# Autodesk Inventor assembly: PCB Stack Concept V03 01
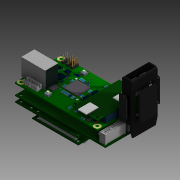
[picture p0: Inventor's stored thumbnail of the model, 180x180]
Saved by Autodesk Inventor 2013 (Build 170138000, 138)
## iProperties
Created: 2014-04-13
Part Number: PCB Stack Concept V03 01
Document SubType Name: Assembly
Designer: spichelh
Author: spichelh
## Documents named in this file (37)
- C:\Users\spichelh\Documents\GitHub\beta-hardware\Enclosure\Version 002\PCB Stack Concept V03 01.iam
- C:\Users\spichelh\Documents\GitHub\beta-hardware\Enclosure\Version 002\Enclosure-Backplate01.ipt
- C:\Users\spichelh\Documents\GitHub\beta-hardware\Enclosure\Version 002\KAC12040.ipt
- C:\Users\spichelh\Documents\GitHub\beta-hardware\Enclosure\Version 002\IRGlass.ipt
- C:\Users\spichelh\Documents\GitHub\beta-hardware\Enclosure\Version 002\Cooler.ipt
- C:\Users\spichelh\Documents\GitHub\beta-hardware\Enclosure\Version 002\Nikon Mount 02.ipt
- C:\Users\spichelh\Documents\GitHub\beta-hardware\Enclosure\Version 002\IOModulePlate01.ipt
- C:\Users\spichelh\Documents\GitHub\beta-hardware\Enclosure\Version 002\PCBModuleLeft01.ipt
- C:\Users\spichelh\Documents\GitHub\beta-hardware\Enclosure\Version 002\IOModulePlate02.ipt
- C:\Users\spichelh\Documents\GitHub\beta-hardware\Enclosure\Version 002\IOModulePlate03.ipt
- C:\Users\spichelh\Documents\GitHub\beta-hardware\Enclosure\Version 002\PCBModuleRight01.ipt
- C:\Users\spichelh\Documents\GitHub\beta-hardware\Enclosure\Version 002\LensBase02.ipt
- C:\Users\spichelh\Documents\GitHub\beta-hardware\Enclosure\Version 002\HexSaver01.ipt
- C:\Users\spichelh\Documents\GitHub\beta-hardware\Enclosure\Version 002\Enclosure03.ipt
- C:\Users\spichelh\Documents\Inventor\Content Center Files\R2013\en-US\ANSI B18.3.1M(1)\ANSI B18.3.1M - M2,5x0,45 x 16(2).ipt
- C:\Users\spichelh\Documents\Inventor\Content Center Files\R2013\en-US\ANSI B18.3.1M(1)\ANSI B18.3.1M - M2,5x0,45 x 35(2).ipt
- C:\Users\spichelh\Documents\GitHub\beta-hardware\Enclosure\Version 002\LensBaseTop01.ipt
- C:\Users\spichelh\Documents\Inventor\Content Center Files\R2013\en-US\ANSI B18.6.3(00)\ANSI B18.6.3 - 3-48 UNC - 0,25(32).ipt
- C:\Users\spichelh\Documents\GitHub\beta-hardware\Enclosure\Version 002\Unmate01.ipt
- C:\Users\spichelh\Documents\GitHub\beta-hardware\Enclosure\Version 002\Parallella.ipt
- C:\Users\spichelh\Documents\GitHub\beta-hardware\Enclosure\Version 002\SFE-Host01.ipt
- C:\Users\spichelh\Documents\GitHub\beta-hardware\Enclosure\Version 002\SFE-ProcessingBoard01.ipt
- C:\Users\spichelh\Documents\GitHub\beta-hardware\Enclosure\Version 002\CMV12000.ipt
- C:\Users\spichelh\Documents\GitHub\beta-hardware\Enclosure\Version 002\Enclosure-Backplate-Variant02.ipt
- C:\Users\spichelh\Documents\GitHub\beta-hardware\Enclosure\Version 002\PCBModuleLeft02.ipt
- C:\Users\spichelh\Documents\GitHub\beta-hardware\Enclosure\Version 002\BetaBoard01.ipt
- C:\Users\spichelh\Documents\GitHub\beta-hardware\Enclosure\Version 002\Imported Components\Zynq_Z010_uZed_F_Prod\Zynq_Z010_uZed_F_Prod.ipt
- C:\Users\spichelh\Documents\GitHub\beta-hardware\Enclosure\Version 002\HighSpeedIOShield01.ipt
- C:\Users\spichelh\Documents\GitHub\beta-hardware\Enclosure\Version 002\AddonPCB01.ipt
- C:\Users\spichelh\Documents\GitHub\beta-hardware\Enclosure\Version 002\Imported Components\PCI-E x1\PCI-E x1.ipt
- C:\Users\spichelh\Desktop\BetaSkeletonV01.ipt
- C:\Users\spichelh\Documents\GitHub\alpha-hardware\Nikon-F-Mount\Imported Components\F-mount to CMV12k-V04\F-mount to CMV12k-V04.ipt
- C:\Users\spichelh\Desktop\Imported Components\User Library-Mini Displayport Molex-sd-105081-001\User Library-Mini Displayport Molex-sd-105081-001.ipt
- C:\Users\spichelh\Documents\GitHub\beta-hardware\Enclosure\Version 002\DictatorEnclosure4.ipt
- C:\Users\spichelh\Documents\GitHub\beta-hardware\Enclosure\Version 002\IO-Shield-Sideplate01.ipt
- C:\Users\spichelh\Documents\Inventor\Content Center Files\R2013\en-US\ANSI B18.6.3(25)\ANSI B18.6.3 - 2-56 UNC - 0,125(5).ipt
- C:\Users\spichelh\Documents\GitHub\beta-hardware\Enclosure\Version 002\IO-Shield-Topplate01.ipt
## Components (55 placed, 36 different names)
1. Enclosure03:1 — Flush:26, Mate:33, Mate:34, Mate:38, Flush:40, Insert:9, Insert:10, Insert:11, Insert:13, Insert:14, Insert:27, Insert:28, Insert:29, Mate:70, Mate:71, Flush:46, Flush:47
2. Enclosure-Backplate01:1 — Mate:38, Flush:40, Mate:75
3. KAC12040:1 — Mate:72
4. IRGlass:1 — Mate:50, Mate:51, Mate:52
5. Cooler:1 — Mate:35, Flush:43, Flush:44, Mate:67, Mate:68, Mate:69
6. Nikon Mount 02:1 — Mate:31, Mate:32, Insert:3, Mate:50, Mate:51, Mate:52, Insert:18, Insert:19, Insert:20, Insert:21
7. LensBase02:1 — Mate:31, Mate:32, Flush:26, Mate:33, Mate:34, Insert:3, Mate:35, Flush:43, Flush:44, Flush:45
8. IOModulePlate01:1 — Insert:13, Insert:14
9. PCBModuleLeft01:1
10. PCBModuleRight01:1
11. IOModulePlate02:1 — Insert:11
12. IOModulePlate03:1 — Insert:9, Insert:10
13. HexSaver01:1
14. HexSaver01:2
15. HexSaver01:3
16. HexSaver01:4
17. Broached Socket Head Cap Screw - Metric M2,5x0,45 x 16:1 — Insert:18
18. Broached Socket Head Cap Screw - Metric M2,5x0,45 x 16:2 — Insert:19
19. Broached Socket Head Cap Screw - Metric M2,5x0,45 x 16:3 — Insert:20
20. Broached Socket Head Cap Screw - Metric M2,5x0,45 x 16:4 — Insert:21
21. LensBaseTop01:1 — Flush:45, Mate:53, Mate:54, Mate:67, Mate:68, Mate:69
22. Cross Recessed 100° Flat Countersunk Head Machine Screw - Type I - Inch 3-48 UNC x 0,25:2 — Mate:53
23. Cross Recessed 100° Flat Countersunk Head Machine Screw - Type I - Inch 3-48 UNC x 0,25:1 — Mate:54
24. Broached Socket Head Cap Screw - Metric M2,5x0,45 x 35:5 — Mate:55, Mate:70, Mate:71
25. Broached Socket Head Cap Screw - Metric M2,5x0,45 x 35:6 — Insert:27, Mate:59
26. Broached Socket Head Cap Screw - Metric M2,5x0,45 x 35:7 — Insert:28, Mate:66
27. Broached Socket Head Cap Screw - Metric M2,5x0,45 x 35:8 — Insert:29, Mate:57
28. Unmate01:1 — Mate:55
29. Unmate01:2 — Mate:57
30. Unmate01:3 — Mate:59
31. Unmate01:4 — Mate:66
32. Parallella:1
33. SFE-Host01:1 — Mate:72, Mate:73, Flush:48, Flush:49, Mate:76, Flush:50, Flush:51, Flush:78
34. SFE-ProcessingBoard01:1 — Mate:73, Flush:48, Flush:49, Mate:77, Flush:85
35. CMV12000:1 — Mate:76, Flush:50, Flush:51, Mate:91, Mate:92, Mate:93
36. Enclosure-Backplate-Variant02:1 — Mate:75, Flush:46, Flush:47
37. PCBModuleLeft02:1 — Flush:52, Flush:79, Mate:79
38. BetaBoard01:1 — Mate:77, Flush:52, Flush:78, Flush:79, Mate:79, Flush:85, Flush:86, Flush:87, Mate:80, Flush:88, Mate:84, Mate:85, Flush:94, Flush:95, Flush:96, Flush:97
39. Zynq_Z010_uZed_F_Prod:1 — Flush:86, Flush:87, Mate:80, Flush:91, Mate:83, Flush:92
40. HighSpeedIOShield01:1 — Flush:88, Mate:86, Mate:87, Mate:97, Mate:98, Mate:99, Flush:100, Mate:100, Mate:102, Mate:103, Mate:104, Mate:113, Mate:114, Mate:115, Mate:116, Mate:117, Mate:118, Mate:119, Mate:120, Mate:121, Mate:122, Mate:123, Mate:124, Mate:125, Mate:126
41. AddonPCB01:1 — Flush:91, Mate:83, Flush:92
42. PCI-E x1:1 — Mate:84, Flush:94, Flush:97, Mate:86, Mate:87
43. PCI-E x1:2 — Mate:85, Flush:95, Flush:96
44. BetaSkeletonV01:1 — Mate:94, Mate:95, Mate:96, Mate:39
45. F-mount to CMV12k-V04:1 — Mate:91, Mate:92, Mate:93, Mate:94, Mate:95, Mate:96
46. User Library-Mini Displayport Molex-sd-105081-001:1 — Mate:99, Flush:100, Mate:101, Mate:102, Flush:101
47. DictatorEnclosure4:1 — Mate:97, Mate:98
48. User Library-Mini Displayport Molex-sd-105081-001:2 — Mate:100, Mate:101, Flush:101
49. IO-Shield-Sideplate01:1 — Mate:103, Mate:104
50. Cross Recessed Pan Head Machine Screw - Type IA - Inch No. 2 - 56 - 1/8:1 — Mate:113, Mate:114
51. Cross Recessed Pan Head Machine Screw - Type IA - Inch No. 2 - 56 - 1/8:2 — Mate:115, Mate:116
52. Cross Recessed Pan Head Machine Screw - Type IA - Inch No. 2 - 56 - 1/8:3 — Mate:117, Mate:118
53. Cross Recessed Pan Head Machine Screw - Type IA - Inch No. 2 - 56 - 1/8:4 — Mate:119, Mate:120
54. IO-Shield-Topplate01:1 — Mate:124, Mate:125, Mate:126
55. IO-Shield-Topplate01:2 — Mate:121, Mate:122, Mate:123
## Relationships (100: Mate 61, Flush 26, Insert 13)
- Mate:31: Nikon Mount 02:1 ↔ LensBase02:1
- Mate:32: Nikon Mount 02:1 ↔ LensBase02:1
- Flush:26: Enclosure03:1 ↔ LensBase02:1
- Mate:33: Enclosure03:1 ↔ LensBase02:1
- Mate:34: Enclosure03:1 ↔ LensBase02:1
- Insert:3: Nikon Mount 02:1 ↔ LensBase02:1
- Mate:35: Cooler:1 ↔ LensBase02:1
- Mate:38 (3 mm): Enclosure03:1 ↔ Enclosure-Backplate01:1
- Flush:40: Enclosure03:1 ↔ Enclosure-Backplate01:1
- Mate:39: BetaSkeletonV01:1
- Insert:9: Enclosure03:1 ↔ IOModulePlate03:1
- Insert:10: Enclosure03:1 ↔ IOModulePlate03:1
- Insert:11: Enclosure03:1 ↔ IOModulePlate02:1
- Insert:13: Enclosure03:1 ↔ IOModulePlate01:1
- Insert:14: Enclosure03:1 ↔ IOModulePlate01:1
- Mate:50: IRGlass:1 ↔ Nikon Mount 02:1
- Mate:51 (0.5 mm): IRGlass:1 ↔ Nikon Mount 02:1
- Mate:52 (0.5 mm): IRGlass:1 ↔ Nikon Mount 02:1
- Flush:43: Cooler:1 ↔ LensBase02:1
- Flush:44: Cooler:1 ↔ LensBase02:1
- Flush:45: LensBase02:1 ↔ LensBaseTop01:1
- Mate:55: Broached Socket Head Cap Screw - Metric M2,5x0,45 x 35:5 ↔ Unmate01:1
- Mate:57: Broached Socket Head Cap Screw - Metric M2,5x0,45 x 35:8 ↔ Unmate01:2
- Mate:59: Broached Socket Head Cap Screw - Metric M2,5x0,45 x 35:6 ↔ Unmate01:3
- Mate:66: Broached Socket Head Cap Screw - Metric M2,5x0,45 x 35:7 ↔ Unmate01:4
- Mate:67: Cooler:1 ↔ LensBaseTop01:1
- Mate:68: Cooler:1 ↔ LensBaseTop01:1
- Mate:69: Cooler:1 ↔ LensBaseTop01:1
- Mate:70: Enclosure03:1 ↔ Broached Socket Head Cap Screw - Metric M2,5x0,45 x 35:5
- Mate:71: Enclosure03:1 ↔ Broached Socket Head Cap Screw - Metric M2,5x0,45 x 35:5
- Mate:72: KAC12040:1 ↔ SFE-Host01:1
- Mate:73: SFE-Host01:1 ↔ SFE-ProcessingBoard01:1
- Mate:75 (10 mm): Enclosure-Backplate01:1 ↔ Enclosure-Backplate-Variant02:1
- Flush:46: Enclosure03:1 ↔ Enclosure-Backplate-Variant02:1
- Flush:47: Enclosure03:1 ↔ Enclosure-Backplate-Variant02:1
- Flush:48: SFE-Host01:1 ↔ SFE-ProcessingBoard01:1
- Flush:49: SFE-Host01:1 ↔ SFE-ProcessingBoard01:1
- Mate:76 (3 mm): SFE-Host01:1 ↔ CMV12000:1
- Flush:50 (6 mm): SFE-Host01:1 ↔ CMV12000:1
- Flush:51 (11.75 mm): SFE-Host01:1 ↔ CMV12000:1
- Mate:77: SFE-ProcessingBoard01:1 ↔ BetaBoard01:1
- Flush:52: PCBModuleLeft02:1 ↔ BetaBoard01:1
- Flush:78: SFE-Host01:1 ↔ BetaBoard01:1
- Flush:79: PCBModuleLeft02:1 ↔ BetaBoard01:1
- Mate:79 (6 mm): PCBModuleLeft02:1 ↔ BetaBoard01:1
- Flush:85 (-21 mm): SFE-ProcessingBoard01:1 ↔ BetaBoard01:1
- Flush:86: BetaBoard01:1 ↔ Zynq_Z010_uZed_F_Prod:1
- Flush:87: BetaBoard01:1 ↔ Zynq_Z010_uZed_F_Prod:1
- Mate:80 (12 mm): BetaBoard01:1 ↔ Zynq_Z010_uZed_F_Prod:1
- Flush:88: BetaBoard01:1 ↔ HighSpeedIOShield01:1
- Flush:91: Zynq_Z010_uZed_F_Prod:1 ↔ AddonPCB01:1
- Mate:83: Zynq_Z010_uZed_F_Prod:1 ↔ AddonPCB01:1
- Flush:92: Zynq_Z010_uZed_F_Prod:1 ↔ AddonPCB01:1
- Mate:84: BetaBoard01:1 ↔ PCI-E x1:1
- Mate:85: BetaBoard01:1 ↔ PCI-E x1:2
- Flush:94 (2 mm): BetaBoard01:1 ↔ PCI-E x1:1
- Flush:95 (2 mm): BetaBoard01:1 ↔ PCI-E x1:2
- Flush:96 (2 mm): BetaBoard01:1 ↔ PCI-E x1:2
- Flush:97 (2 mm): BetaBoard01:1 ↔ PCI-E x1:1
- Mate:86: HighSpeedIOShield01:1 ↔ PCI-E x1:1
- Mate:87: HighSpeedIOShield01:1 ↔ PCI-E x1:1
- Mate:91: CMV12000:1 ↔ F-mount to CMV12k-V04:1
- Mate:92: CMV12000:1 ↔ F-mount to CMV12k-V04:1
- Mate:93: CMV12000:1 ↔ F-mount to CMV12k-V04:1
- Mate:94: BetaSkeletonV01:1 ↔ F-mount to CMV12k-V04:1
- Mate:95: BetaSkeletonV01:1 ↔ F-mount to CMV12k-V04:1
- Mate:96: BetaSkeletonV01:1 ↔ F-mount to CMV12k-V04:1
- Mate:97: HighSpeedIOShield01:1 ↔ DictatorEnclosure4:1
- Mate:98: HighSpeedIOShield01:1 ↔ DictatorEnclosure4:1
- Mate:99: HighSpeedIOShield01:1 ↔ User Library-Mini Displayport Molex-sd-105081-001:1
- Flush:100 (4 mm): HighSpeedIOShield01:1 ↔ User Library-Mini Displayport Molex-sd-105081-001:1
- Mate:100: HighSpeedIOShield01:1 ↔ User Library-Mini Displayport Molex-sd-105081-001:2
- Mate:101 (2 mm): User Library-Mini Displayport Molex-sd-105081-001:1 ↔ User Library-Mini Displayport Molex-sd-105081-001:2
- Mate:102 (1 mm): HighSpeedIOShield01:1 ↔ User Library-Mini Displayport Molex-sd-105081-001:1
- Flush:101: User Library-Mini Displayport Molex-sd-105081-001:1 ↔ User Library-Mini Displayport Molex-sd-105081-001:2
- Mate:103 (5 mm): HighSpeedIOShield01:1 ↔ IO-Shield-Sideplate01:1
- Mate:104: HighSpeedIOShield01:1 ↔ IO-Shield-Sideplate01:1
- Mate:114: HighSpeedIOShield01:1 ↔ Cross Recessed Pan Head Machine Screw - Type IA - Inch No. 2 - 56 - 1/8:1
- Mate:116: HighSpeedIOShield01:1 ↔ Cross Recessed Pan Head Machine Screw - Type IA - Inch No. 2 - 56 - 1/8:2
- Mate:118: HighSpeedIOShield01:1 ↔ Cross Recessed Pan Head Machine Screw - Type IA - Inch No. 2 - 56 - 1/8:3
- Mate:120: HighSpeedIOShield01:1 ↔ Cross Recessed Pan Head Machine Screw - Type IA - Inch No. 2 - 56 - 1/8:4
- Mate:121: HighSpeedIOShield01:1 ↔ IO-Shield-Topplate01:2
- Mate:122: HighSpeedIOShield01:1 ↔ IO-Shield-Topplate01:2
- Mate:123 (5 mm): HighSpeedIOShield01:1 ↔ IO-Shield-Topplate01:2
- Mate:124: HighSpeedIOShield01:1 ↔ IO-Shield-Topplate01:1
- Mate:125: HighSpeedIOShield01:1 ↔ IO-Shield-Topplate01:1
- Mate:126 (5 mm): HighSpeedIOShield01:1 ↔ IO-Shield-Topplate01:1
- Insert:18: Nikon Mount 02:1 ↔ Broached Socket Head Cap Screw - Metric M2,5x0,45 x 16:1
- Insert:19: Nikon Mount 02:1 ↔ Broached Socket Head Cap Screw - Metric M2,5x0,45 x 16:2
- Insert:20: Nikon Mount 02:1 ↔ Broached Socket Head Cap Screw - Metric M2,5x0,45 x 16:3
- Insert:21: Nikon Mount 02:1 ↔ Broached Socket Head Cap Screw - Metric M2,5x0,45 x 16:4
- Mate:53: LensBaseTop01:1 ↔ Cross Recessed 100° Flat Countersunk Head Machine Screw - Type I - Inch 3-48 UNC x 0,25:2
- Mate:54: LensBaseTop01:1 ↔ Cross Recessed 100° Flat Countersunk Head Machine Screw - Type I - Inch 3-48 UNC x 0,25:1
- Insert:27: Enclosure03:1 ↔ Broached Socket Head Cap Screw - Metric M2,5x0,45 x 35:6
- Insert:28: Enclosure03:1 ↔ Broached Socket Head Cap Screw - Metric M2,5x0,45 x 35:7
- Insert:29: Enclosure03:1 ↔ Broached Socket Head Cap Screw - Metric M2,5x0,45 x 35:8
- Mate:113: HighSpeedIOShield01:1 ↔ Cross Recessed Pan Head Machine Screw - Type IA - Inch No. 2 - 56 - 1/8:1
- Mate:115: HighSpeedIOShield01:1 ↔ Cross Recessed Pan Head Machine Screw - Type IA - Inch No. 2 - 56 - 1/8:2
- Mate:117: HighSpeedIOShield01:1 ↔ Cross Recessed Pan Head Machine Screw - Type IA - Inch No. 2 - 56 - 1/8:3
- Mate:119: HighSpeedIOShield01:1 ↔ Cross Recessed Pan Head Machine Screw - Type IA - Inch No. 2 - 56 - 1/8:4
